# Autodesk Inventor assembly: MCGS16-5-8
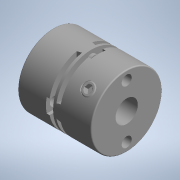
[picture p0: Inventor's stored thumbnail of the model, 180x180]
Saved by Autodesk Inventor 2022.3 (Build 263350000, 350)
## iProperties
Part Number: MCGS16-5-8
Catalog Web Link: www.cadenas.de
Description: MCGS, MCGSRK, MCGSWK-Couplings - Standard Torque, Set Screw Type - Single Disk Type
Vendor: MISUMI
Document SubType Name: Assembly
Designer: partserver
Manufacturer: MISUMI
Mass: 2.35939 g
Surface Area: 24.5452 cm^2
Volume: 2.35939 cm^3
Density: 1 g/cm^3
Category: PARTsolutions
Company: MISUMI
PSOL_IDENT_0: {$CADENAS_DATA\23d-libs\misumi\metric\50_couplings\mcgsrk_asmtab.prj},231 {VTYP=3D},{STYP=ASSTAB},{N
PSOL_IDENT_1: B=MCGS16-5-8},{LINA=MCGS16-5-8},{NN=MCGS, MCGSRK, MCGSWK},{DATE=08.06.2021 06:32:33},{GEOMDATE=27.08
PSOL_IDENT_2: .2013},{VERSION=},{LINEID=1040},{WBVAR=HS,KGHS,DD1,ALT1,LDC,DD2,ALT2,RDC,ALT3,ALT4},{WBNUMERIC=LDC,R
PSOL_IDENT_3: DC}  {NB=MCGS16-5-8},{LINA=MCGS16-5-8},{KT=DUMMY},{PN=MCGS16-5-8},{HS=MCGS},{HSALG='MCGS','Standard
PSOL_IDENT_4: Hole','','Key Groove Hole'},{KGHS=},{KGHSALG='','N/A'},{MATB=Aluminum Die Casting},{MATD=Polyimid},{
PSOL_IDENT_5: STB=Electroless Nickel Plating},{AC=Set Screw},{D=16},{DDIA=16.000},{D1='4','4','5','5','6','6','6.3
PSOL_IDENT_6: 5','6.35','7','7','8','8'},{DD1=5},{DD1ALG1='4','4','5','5','6','6','6.35','6.35','7','7','8','8'},{
PSOL_IDENT_7: DD1ALG2=5},{ALT1=},{ALT1ALG=},{LDC=0.0},{LDCALG=0},{LDCALG1=},{LK=0},{D2='5','5','6','6','6.35','6.3
PSOL_IDENT_8: 5','7','7','8','8'},{DD2=8},{DDD1=5},{DD2ALG1='5','5','6','6','6.35','6.35','7','7','8','8'},{DD2ALG
PSOL_IDENT_9: 11='4','4','5','5','6','6','6.35','6.35','7','7','8','8'},{DD2ALG2=8},{ALT2=},{ALT2ALG=},{RDC=0.0},{
PSOL_IDENT_10: RDCALG=0},{RDCALG1=},{RK=0},{DD3=6.8},{L=16.5},{L1=16.500},{LL=7},{LL1=7.000},{F=3},{F1=3.000},{M=M3
PSOL_IDENT_11: },{T=0.7},{NO=3},{DDIA2=11.2014},{SC1=1.7500},{SC2=6.0000},{DL=5},{TSIMD=3.000},{DR=8},{TSIMIN=2.459
PSOL_IDENT_12: },{ALTALG2='','Select RDC'},{TSI=M3},{R1=2.250},{DDIA3=12.000},{LL2=0.950},{C=3.000},{B=3.500},{E=3.
PSOL_IDENT_13: 200},{F2=0.650},{LL3=4.400},{DDIA4=9.000},{TSIMD1=4.800},{TTL=0.0},{TTR=0.0},{ALT3=},{ALT3ALG= '', '
PSOL_IDENT_14: N/A'},{ALT3PN=},{ALT4=},{ALT4ALG= '', 'N/A'},{ALT4PN=},{KLH=0},{KRH=2},{TTKLH=0.0},{TTKRH=1.0},{MSS=
PSOL_IDENT_15: 3},{LSS=4},{PPATH=mcgs_asmtpl.prj},{DID=7.6}
NB: MCGS16-5-8
NN: MCGS, MCGSRK, MCGSWK
NT: Couplings - Standard Torque, Set Screw Type - Single Disk Type
NBSYN: $PN.
LINA: MCGS16-5-8
CATALOG: Misumi
PN: MCGS16-5-8
HS: Standard Hole
KGHS: N/A
MATB: Aluminum Die Casting
MATD: Polyimid
STB: Electroless Nickel Plating
AC: Set Screw
D: 16
DD1: 5
ALT1: w/o LDC (Shaft Hole Diameter Left Shaft)
LDC: 0
DD2: 8
ALT2: w/o RDC (Shaft Hole Diameter Right Shaft)
RDC: 0
L: 16.5
LL: 7
F: 3
M: M3
T: 0.7
ALT3: N/A
ALT4: N/A
SUPPLIER: MISUMI
ARTICLENO: MCGS16-5-8
BOMINFO: MCGS16-5-8
CREATOR: CADENAS GmbH
Title: MCGS16-5-8
Author: Cadenas PARTsolutions
Comments: Couplings - Standard Torque, Set Screw Type - Single Disk Type
## Documents named in this file (3)
- C:\Users\YusukeKunita\Documents\GrabCAD\Development\BasicParts\Coupling\MCGS16-5-8\MCGS16-5-8.iam
- C:\Users\YusukeKunita\Documents\GrabCAD\Development\BasicParts\Coupling\MCGS16-5-8\MCGS16-5-8_b.ipt
- C:\Users\YusukeKunita\Documents\GrabCAD\Development\BasicParts\Coupling\MCGS16-5-8\Hexagon socket set screw with flat point DIN 913 - M3x4.ipt
## Components (5 placed, 2 different names)
1. MCGS16-5-8_b:1 — to_screw1_Z@1 <-> IP1_Z@2, to_screw2_Z@1 <-> IP1_Z@3, to_screw3_Z@1 <-> IP1_Z@4, to_screw4_Z@1 <-> IP1_Z@5
2. Hexagon socket set screw with flat point DIN 913 - M3x4:1 — to_screw1_Z@1 <-> IP1_Z@2
3. Hexagon socket set screw with flat point DIN 913 - M3x4:2 — to_screw2_Z@1 <-> IP1_Z@3
4. Hexagon socket set screw with flat point DIN 913 - M3x4:3 — to_screw3_Z@1 <-> IP1_Z@4
5. Hexagon socket set screw with flat point DIN 913 - M3x4:4 — to_screw4_Z@1 <-> IP1_Z@5
## Relationships (4: Mate 4)
- to_screw1_Z@1 <-> IP1_Z@2 [Mate]: MCGS16-5-8_b:1 ↔ Hexagon socket set screw with flat point DIN 913 - M3x4:1
- to_screw2_Z@1 <-> IP1_Z@3 [Mate]: MCGS16-5-8_b:1 ↔ Hexagon socket set screw with flat point DIN 913 - M3x4:2
- to_screw3_Z@1 <-> IP1_Z@4 [Mate]: MCGS16-5-8_b:1 ↔ Hexagon socket set screw with flat point DIN 913 - M3x4:3
- to_screw4_Z@1 <-> IP1_Z@5 [Mate]: MCGS16-5-8_b:1 ↔ Hexagon socket set screw with flat point DIN 913 - M3x4:4
